# Autodesk Inventor assembly: ARDUINO PRO MICROCool
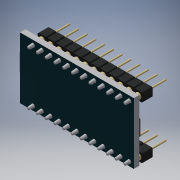
[picture p0: Inventor's stored thumbnail of the model, 180x180]
Saved by Autodesk Inventor 2018 (Build 220112000, 112)
## iProperties
Created: 2015-09-14
Part Number: ARDUINO PRO MICROCool
Material: Generisch
Description: STEP AP214
Document SubType Name: Assembly
Designer: Markus
Title: ARDUINO PRO MICRO.STEP
Author: A
Revision Number: ANY
Sending System: SolidWorks 2014
Preprocessor: SwSTEP 2.0
## Documents named in this file (16)
- G:\VolumeKnob\Objekts\ARDUINO PRO MICROCool.iam
- G:\VolumeKnob\Objekts\micro board.ipt
- G:\VolumeKnob\Objekts\MICRO_stackable header 12.iam
- G:\VolumeKnob\Objekts\micro usb.iam
- G:\VolumeKnob\Objekts\atmega32U4.ipt
- G:\VolumeKnob\Objekts\MICRO_cap106C.ipt
- G:\VolumeKnob\Objekts\micro_crystal 5x3.ipt
- G:\VolumeKnob\Objekts\micro_MIC5219.ipt
- G:\VolumeKnob\Objekts\MICRO_603 resistor 103.ipt
- G:\VolumeKnob\Objekts\MICRO_603 resistor 102.ipt
- G:\VolumeKnob\Objekts\MICRO_603 resistor 22.ipt
- G:\VolumeKnob\Objekts\MICRO_PTC-1206.ipt
- G:\VolumeKnob\Objekts\MICRO_603 resistor 331.ipt
- G:\VolumeKnob\Objekts\MICRO_603 cap on pad.ipt
- G:\VolumeKnob\Objekts\SOD 323.ipt
- G:\VolumeKnob\Objekts\MICRO_led.ipt
## Components (27 placed, 27 different names)
1. micro board_1 — Passend:1, Passend:2, Passend:3, Passend:4
2. MICRO_stackable header 12_2 [sub-assembly] — Passend:3, Passend:4
3. micro usb_3 [sub-assembly]
4. atmega32U4_4
5. MICRO_cap106C_5
6. MICRO_cap106C_6
7. MICRO_stackable header 12_7 [sub-assembly] — Passend:1, Passend:2
8. micro_crystal 5x3_8
9. micro_MIC5219_9
10. MICRO_603 resistor 103_10
11. MICRO_603 resistor 102_11
12. MICRO_603 resistor 22_12
13. MICRO_603 resistor 22_13
14. MICRO_PTC-1206_14
15. MICRO_603 resistor 331_15
16. MICRO_603 resistor 331_16
17. MICRO_603 cap on pad_17
18. MICRO_603 cap on pad_18
19. MICRO_603 cap on pad_19
20. MICRO_603 cap on pad_20
21. MICRO_603 cap on pad_21
22. MICRO_603 cap on pad_22
23. MICRO_603 cap on pad_23
24. SOD 323_24
25. MICRO_led_25
26. MICRO_led_26
27. MICRO_led_27
## Relationships (4: Mate 4)
- Passend:1 [Mate]: micro board_1 ↔ MICRO_stackable header 12_7
- Passend:2 [Mate]: micro board_1 ↔ MICRO_stackable header 12_7
- Passend:3 [Mate]: micro board_1 ↔ MICRO_stackable header 12_2
- Passend:4 [Mate]: micro board_1 ↔ MICRO_stackable header 12_2
